# Autodesk Inventor assembly: capsule.bottom.assembly
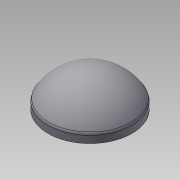
[picture p0: Inventor's stored thumbnail of the model, 180x180]
Saved by Autodesk Inventor 2011 (Build 150239000, 239)
## iProperties
Created: 2011-01-27
Part Number: capsule.bottom.assembly
Document SubType Name: Assembly
Designer: Casey
Author: Casey
## Documents named in this file (6)
- C:\Users\Casey\Documents\My Dropbox\RockSAT-X 2011 RexSAT\capsule-launcher.design\Capsule\capsule.bottom.assembly.iam
- C:\Users\Casey\Documents\My Dropbox\RockSAT-X 2011 RexSAT\capsule-launcher.design\Capsule\Capsule.bottom.ipt
- C:\Users\Casey\Documents\My Dropbox\RockSAT-X 2011 RexSAT\capsule-launcher.design\Capsule\capsule.electronics.board.ipt
- C:\Users\Casey\Documents\My Dropbox\RockSAT-X 2011 RexSAT\capsule-launcher.design\Capsule\capsule.gasket.ipt
- C:\Users\Casey\Documents\My Dropbox\RockSAT-X 2011 RexSAT\capsule-launcher.design\Capsule\3mm-standoff-16-long.ipt
- C:\Users\Casey\Documents\My Dropbox\RockSAT-X 2011 RexSAT\capsule-launcher.design\ANSI B18.3.1M(6)\ANSI B18.3.1M - M3x0.5 x 5(1).ipt
## Components (16 placed, 5 different names)
1. Capsule.bottom:1 — Mate:1, Mate:2, Mate:3, Mate:4, Mate:5, Mate:6, Mate:7
2. capsule.electronics.board:1 — Mate:1, Mate:2, Mate:3, Insert:1
3. capsule.gasket:1 — Mate:4, Mate:5, Mate:6
4. capsule.electronics.board:2 — Mate:7, Mate:8, Mate:9, Insert:2, Insert:3, Insert:4, Insert:5, Insert:6, Insert:7
5. Forged Socket Head Cap Screw - Metric M3x0.5 x 5:1 — Insert:2
6. Forged Socket Head Cap Screw - Metric M3x0.5 x 5:2 — Insert:3
7. Forged Socket Head Cap Screw - Metric M3x0.5 x 5:3 — Insert:4
8. Forged Socket Head Cap Screw - Metric M3x0.5 x 5:4 — Insert:5
9. Forged Socket Head Cap Screw - Metric M3x0.5 x 5:5 — Insert:6
10. Forged Socket Head Cap Screw - Metric M3x0.5 x 5:6 — Insert:7
11. 3mm-standoff-16-long:1 — Insert:1
12. 3mm-standoff-16-long:2
13. 3mm-standoff-16-long:3
14. 3mm-standoff-16-long:4
15. 3mm-standoff-16-long:5
16. 3mm-standoff-16-long:6 — Mate:8, Mate:9
## Component patterns: (6 elements, first: 3mm-standoff-16-long:1)
## Relationships (16: Mate 9, Insert 7)
- Mate:1: Capsule.bottom:1 ↔ capsule.electronics.board:1
- Mate:2: Capsule.bottom:1 ↔ capsule.electronics.board:1
- Mate:3: Capsule.bottom:1 ↔ capsule.electronics.board:1
- Mate:4: Capsule.bottom:1 ↔ capsule.gasket:1
- Mate:5: Capsule.bottom:1 ↔ capsule.gasket:1
- Mate:6: Capsule.bottom:1 ↔ capsule.gasket:1
- Insert:1: capsule.electronics.board:1 ↔ 3mm-standoff-16-long:1
- Mate:7: Capsule.bottom:1 ↔ capsule.electronics.board:2
- Mate:8: capsule.electronics.board:2 ↔ 3mm-standoff-16-long:6
- Mate:9: capsule.electronics.board:2 ↔ 3mm-standoff-16-long:6
- Insert:2: capsule.electronics.board:2 ↔ Forged Socket Head Cap Screw - Metric M3x0.5 x 5:1
- Insert:3: capsule.electronics.board:2 ↔ Forged Socket Head Cap Screw - Metric M3x0.5 x 5:2
- Insert:4: capsule.electronics.board:2 ↔ Forged Socket Head Cap Screw - Metric M3x0.5 x 5:3
- Insert:5: capsule.electronics.board:2 ↔ Forged Socket Head Cap Screw - Metric M3x0.5 x 5:4
- Insert:6: capsule.electronics.board:2 ↔ Forged Socket Head Cap Screw - Metric M3x0.5 x 5:5
- Insert:7: capsule.electronics.board:2 ↔ Forged Socket Head Cap Screw - Metric M3x0.5 x 5:6
